# Autodesk Inventor assembly: Assembly
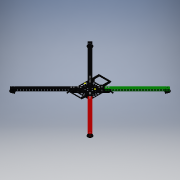
[picture p0: Inventor's stored thumbnail of the model, 180x180]
Saved by Autodesk Inventor 2016 (Build 200138000, 138)
## iProperties
Created: 2016-03-06
Part Number: Assembly
Document SubType Name: Assembly
Designer: dimas
Author: dimas
## Documents named in this file (10)
- C:\Users\dimas\Documents\lap_quad\Assembly.iam
- C:\Users\dimas\Documents\lap_quad\Arm_light.ipt
- C:\Users\dimas\Documents\lap_quad\frame_mount.ipt
- C:\Users\dimas\Documents\lap_quad\plate_mk2.ipt
- C:\Users\dimas\Documents\lap_quad\motor_mount.ipt
- C:\Users\dimas\Documents\lap_quad\battery_clip.ipt
- C:\Users\dimas\Documents\Inventor\Content Center Files\R2016\en-US\ANSI B18.3.1M(6)\ANSI B18.3.1M - M3x0.5 x 25(1).ipt
- C:\Users\dimas\Documents\Inventor\Content Center Files\R2016\en-US\AS 1971 (M - 6)\AS 1971 - 3.5(2).ipt
- C:\Users\dimas\Documents\Inventor\Content Center Files\R2016\en-US\AS 1112 (2)\AS 1112 - M3  Type 5.ipt
- C:\Users\dimas\Documents\Inventor\Content Center Files\R2016\en-US\AS 1112 (2)\AS 1112 - M3  Type 8.ipt
## Components (56 placed, 9 different names)
1. Arm_light:1 — Mate:1, Mate:2, Flush:1, Mate:25, Mate:26, Mate:27, Mate:40, Mate:41, Mate:66, Mate:67
2. frame_mount:1 — Mate:1, Mate:2, Flush:1, Mate:3, Mate:4, Flush:2, Mate:5, Mate:6, Flush:3, Mate:73, Mate:75
3. plate_mk2:1 — Mate:3, Mate:4, Flush:2, Mate:7, Mate:8, Mate:9, Mate:10, Mate:11, Mate:12, Mate:13, Mate:14, Mate:15, Flush:7, Flush:8, Flush:9, Mate:34, Mate:35, Mate:36, Mate:37, Mate:38, Mate:39, Mate:49, Mate:51, Mate:53, Mate:55, Mate:68, Mate:69, Mate:70, Mate:71
4. plate_mk2:2 — Mate:5, Mate:6, Flush:3, Mate:96
5. frame_mount:2 — Mate:7, Mate:8, Mate:9, Mate:16, Mate:17, Flush:4, Mate:77, Mate:79
6. frame_mount:3 — Mate:13, Mate:14, Mate:15, Mate:20, Mate:21, Flush:6, Mate:81, Mate:83
7. frame_mount:4 — Mate:10, Mate:11, Mate:12, Mate:18, Mate:19, Flush:5, Mate:85, Mate:87
8. Arm_light:2 — Mate:16, Mate:17, Flush:4, Mate:28, Mate:29, Mate:30, Mate:42, Mate:43, Mate:57, Mate:58
9. Arm_light:3 — Mate:18, Mate:19, Flush:5, Mate:31, Mate:32, Mate:33, Mate:46, Mate:47, Mate:63, Mate:64
10. Arm_light:4 — Mate:20, Mate:21, Flush:6, Mate:22, Mate:23, Mate:24, Mate:44, Mate:45, Mate:60, Mate:61
11. motor_mount:1 — Mate:22, Mate:23, Mate:24
12. motor_mount:2 — Mate:25, Mate:26, Mate:27
13. motor_mount:3 — Mate:28, Mate:29, Mate:30
14. motor_mount:4 — Mate:31, Mate:32, Mate:33
15. battery_clip:1 — Mate:34, Mate:35, Mate:36, Mate:48, Mate:54, Mate:59, Mate:62
16. battery_clip:2 — Mate:37, Mate:38, Mate:39, Mate:50, Mate:52, Mate:56, Mate:65
17. Forged Socket Head Cap Screw - Metric M3x0.5 x 25:1 — Mate:44, Mate:60, Mate:80, Mate:99
18. Forged Socket Head Cap Screw - Metric M3x0.5 x 25:2 — Mate:45, Mate:61, Mate:82, Mate:100
19. Forged Socket Head Cap Screw - Metric M3x0.5 x 25:3 — Mate:46, Mate:64, Mate:86, Mate:106
20. Forged Socket Head Cap Screw - Metric M3x0.5 x 25:4 — Mate:47, Mate:63, Mate:84, Mate:105
21. Forged Socket Head Cap Screw - Metric M3x0.5 x 25:5 — Mate:40, Mate:67, Mate:74, Mate:89
22. Forged Socket Head Cap Screw - Metric M3x0.5 x 25:6 — Mate:41, Mate:66, Mate:72, Mate:91
23. Forged Socket Head Cap Screw - Metric M3x0.5 x 25:7 — Mate:42, Mate:58, Mate:78, Mate:92
24. Forged Socket Head Cap Screw - Metric M3x0.5 x 25:8 — Mate:43, Mate:57, Mate:76, Mate:93
25. Forged Socket Head Cap Screw - Metric M3x0.5 x 25:9 — Mate:48, Mate:62, Mate:101
26. Forged Socket Head Cap Screw - Metric M3x0.5 x 25:10 — Mate:50, Mate:65, Mate:103
27. Forged Socket Head Cap Screw - Metric M3x0.5 x 25:11 — Mate:51, Mate:71, Mate:104
28. Forged Socket Head Cap Screw - Metric M3x0.5 x 25:12 — Mate:52, Mate:56, Mate:97
29. Forged Socket Head Cap Screw - Metric M3x0.5 x 25:13 — Mate:49, Mate:70, Mate:102
30. Forged Socket Head Cap Screw - Metric M3x0.5 x 25:14 — Mate:54, Mate:59, Mate:94
31. Forged Socket Head Cap Screw - Metric M3x0.5 x 25:15 — Mate:55, Mate:68, Mate:95
32. Forged Socket Head Cap Screw - Metric M3x0.5 x 25:16 — Mate:53, Mate:69, Mate:98
33. AS 1971 (M - 6) 3.5:1 — Mate:72, Mate:73
34. AS 1971 (M - 6) 3.5:2 — Mate:74, Mate:75, Mate:90
35. AS 1971 (M - 6) 3.5:3 — Mate:76, Mate:77
36. AS 1971 (M - 6) 3.5:4 — Mate:78, Mate:79
37. AS 1971 (M - 6) 3.5:5 — Mate:80, Mate:81
38. AS 1971 (M - 6) 3.5:6 — Mate:82, Mate:83
39. AS 1971 (M - 6) 3.5:7 — Mate:84, Mate:85
40. AS 1971 (M - 6) 3.5:8 — Mate:86, Mate:87
41. AS 1112 (2) - Metric M3  Type 5:1 — Mate:89, Mate:90, Flush:10, Flush:11, Flush:12, Flush:18
42. AS 1112 (2) - Metric M3  Type 8:1 — Mate:93, Flush:12
43. AS 1112 (2) - Metric M3  Type 8:2 — Mate:92, Flush:11
44. AS 1112 (2) - Metric M3  Type 8:3 — Mate:95, Flush:13, Flush:14, Flush:17
45. AS 1112 (2) - Metric M3  Type 8:4 — Mate:94, Mate:96, Flush:13, Flush:15, Flush:16
46. AS 1112 (2) - Metric M3  Type 8:5 — Mate:98, Flush:14
47. AS 1112 (2) - Metric M3  Type 8:6 — Mate:97, Flush:15
48. AS 1112 (2) - Metric M3  Type 8:7 — Mate:104, Flush:22, Flush:23
49. AS 1112 (2) - Metric M3  Type 8:8 — Mate:103, Flush:23
50. AS 1112 (2) - Metric M3  Type 8:9 — Mate:106, Flush:21
51. AS 1112 (2) - Metric M3  Type 8:10 — Mate:105, Flush:20, Flush:21
52. AS 1112 (2) - Metric M3  Type 8:11 — Mate:100, Flush:18, Flush:19, Flush:20
53. AS 1112 (2) - Metric M3  Type 8:12 — Mate:102, Flush:17, Flush:22
54. AS 1112 (2) - Metric M3  Type 8:13 — Mate:99, Flush:19
55. AS 1112 (2) - Metric M3  Type 8:14 — Mate:101, Flush:16
56. AS 1112 (2) - Metric M3  Type 8:15 — Mate:91, Flush:10
## Relationships (128: Mate 105, Flush 23)
- Mate:1: Arm_light:1 ↔ frame_mount:1
- Mate:2: Arm_light:1 ↔ frame_mount:1
- Flush:1: Arm_light:1 ↔ frame_mount:1
- Mate:3: frame_mount:1 ↔ plate_mk2:1
- Mate:4: frame_mount:1 ↔ plate_mk2:1
- Flush:2: frame_mount:1 ↔ plate_mk2:1
- Mate:5: frame_mount:1 ↔ plate_mk2:2
- Mate:6: frame_mount:1 ↔ plate_mk2:2
- Flush:3: frame_mount:1 ↔ plate_mk2:2
- Mate:7: plate_mk2:1 ↔ frame_mount:2
- Mate:8: plate_mk2:1 ↔ frame_mount:2
- Mate:9: plate_mk2:1 ↔ frame_mount:2
- Mate:10: plate_mk2:1 ↔ frame_mount:4
- Mate:11: plate_mk2:1 ↔ frame_mount:4
- Mate:12: plate_mk2:1 ↔ frame_mount:4
- Mate:13: plate_mk2:1 ↔ frame_mount:3
- Mate:14: plate_mk2:1 ↔ frame_mount:3
- Mate:15: plate_mk2:1 ↔ frame_mount:3
- Mate:16: frame_mount:2 ↔ Arm_light:2
- Mate:17: frame_mount:2 ↔ Arm_light:2
- Flush:4: frame_mount:2 ↔ Arm_light:2
- Mate:18: frame_mount:4 ↔ Arm_light:3
- Mate:19: frame_mount:4 ↔ Arm_light:3
- Flush:5: frame_mount:4 ↔ Arm_light:3
- Mate:20: frame_mount:3 ↔ Arm_light:4
- Mate:21: frame_mount:3 ↔ Arm_light:4
- Flush:6: frame_mount:3 ↔ Arm_light:4
- Flush:7: plate_mk2:1
- Flush:8: plate_mk2:1
- Flush:9: plate_mk2:1
- Mate:22: Arm_light:4 ↔ motor_mount:1
- Mate:23: Arm_light:4 ↔ motor_mount:1
- Mate:24: Arm_light:4 ↔ motor_mount:1
- Mate:25: Arm_light:1 ↔ motor_mount:2
- Mate:26: Arm_light:1 ↔ motor_mount:2
- Mate:27: Arm_light:1 ↔ motor_mount:2
- Mate:28: Arm_light:2 ↔ motor_mount:3
- Mate:29: Arm_light:2 ↔ motor_mount:3
- Mate:30: Arm_light:2 ↔ motor_mount:3
- Mate:31: Arm_light:3 ↔ motor_mount:4
- Mate:32: Arm_light:3 ↔ motor_mount:4
- Mate:33: Arm_light:3 ↔ motor_mount:4
- Mate:34: plate_mk2:1 ↔ battery_clip:1
- Mate:35: plate_mk2:1 ↔ battery_clip:1
- Mate:36: plate_mk2:1 ↔ battery_clip:1
- Mate:37: plate_mk2:1 ↔ battery_clip:2
- Mate:38: plate_mk2:1 ↔ battery_clip:2
- Mate:39: plate_mk2:1 ↔ battery_clip:2
- Mate:40: Arm_light:1 ↔ Forged Socket Head Cap Screw - Metric M3x0.5 x 25:5
- Mate:41: Arm_light:1 ↔ Forged Socket Head Cap Screw - Metric M3x0.5 x 25:6
- Mate:42: Arm_light:2 ↔ Forged Socket Head Cap Screw - Metric M3x0.5 x 25:7
- Mate:43: Arm_light:2 ↔ Forged Socket Head Cap Screw - Metric M3x0.5 x 25:8
- Mate:44: Arm_light:4 ↔ Forged Socket Head Cap Screw - Metric M3x0.5 x 25:1
- Mate:45: Arm_light:4 ↔ Forged Socket Head Cap Screw - Metric M3x0.5 x 25:2
- Mate:46: Arm_light:3 ↔ Forged Socket Head Cap Screw - Metric M3x0.5 x 25:3
- Mate:47: Arm_light:3 ↔ Forged Socket Head Cap Screw - Metric M3x0.5 x 25:4
- Mate:48: battery_clip:1 ↔ Forged Socket Head Cap Screw - Metric M3x0.5 x 25:9
- Mate:49: plate_mk2:1 ↔ Forged Socket Head Cap Screw - Metric M3x0.5 x 25:13
- Mate:50: battery_clip:2 ↔ Forged Socket Head Cap Screw - Metric M3x0.5 x 25:10
- Mate:51: plate_mk2:1 ↔ Forged Socket Head Cap Screw - Metric M3x0.5 x 25:11
- Mate:52: battery_clip:2 ↔ Forged Socket Head Cap Screw - Metric M3x0.5 x 25:12
- Mate:53: plate_mk2:1 ↔ Forged Socket Head Cap Screw - Metric M3x0.5 x 25:16
- Mate:54: battery_clip:1 ↔ Forged Socket Head Cap Screw - Metric M3x0.5 x 25:14
- Mate:55: plate_mk2:1 ↔ Forged Socket Head Cap Screw - Metric M3x0.5 x 25:15
- Mate:56: battery_clip:2 ↔ Forged Socket Head Cap Screw - Metric M3x0.5 x 25:12
- Mate:57: Arm_light:2 ↔ Forged Socket Head Cap Screw - Metric M3x0.5 x 25:8
- Mate:58: Arm_light:2 ↔ Forged Socket Head Cap Screw - Metric M3x0.5 x 25:7
- Mate:59: battery_clip:1 ↔ Forged Socket Head Cap Screw - Metric M3x0.5 x 25:14
- Mate:60: Arm_light:4 ↔ Forged Socket Head Cap Screw - Metric M3x0.5 x 25:1
- Mate:61: Arm_light:4 ↔ Forged Socket Head Cap Screw - Metric M3x0.5 x 25:2
- Mate:62: battery_clip:1 ↔ Forged Socket Head Cap Screw - Metric M3x0.5 x 25:9
- Mate:63: Arm_light:3 ↔ Forged Socket Head Cap Screw - Metric M3x0.5 x 25:4
- Mate:64: Arm_light:3 ↔ Forged Socket Head Cap Screw - Metric M3x0.5 x 25:3
- Mate:65: battery_clip:2 ↔ Forged Socket Head Cap Screw - Metric M3x0.5 x 25:10
- Mate:66: Arm_light:1 ↔ Forged Socket Head Cap Screw - Metric M3x0.5 x 25:6
- Mate:67: Arm_light:1 ↔ Forged Socket Head Cap Screw - Metric M3x0.5 x 25:5
- Mate:68: plate_mk2:1 ↔ Forged Socket Head Cap Screw - Metric M3x0.5 x 25:15
- Mate:69: plate_mk2:1 ↔ Forged Socket Head Cap Screw - Metric M3x0.5 x 25:16
- Mate:70: plate_mk2:1 ↔ Forged Socket Head Cap Screw - Metric M3x0.5 x 25:13
- Mate:71: plate_mk2:1 ↔ Forged Socket Head Cap Screw - Metric M3x0.5 x 25:11
- Mate:72: Forged Socket Head Cap Screw - Metric M3x0.5 x 25:6 ↔ AS 1971 (M - 6) 3.5:1
- Mate:73: frame_mount:1 ↔ AS 1971 (M - 6) 3.5:1
- Mate:74: Forged Socket Head Cap Screw - Metric M3x0.5 x 25:5 ↔ AS 1971 (M - 6) 3.5:2
- Mate:75: frame_mount:1 ↔ AS 1971 (M - 6) 3.5:2
- Mate:76: Forged Socket Head Cap Screw - Metric M3x0.5 x 25:8 ↔ AS 1971 (M - 6) 3.5:3
- Mate:77: frame_mount:2 ↔ AS 1971 (M - 6) 3.5:3
- Mate:78: Forged Socket Head Cap Screw - Metric M3x0.5 x 25:7 ↔ AS 1971 (M - 6) 3.5:4
- Mate:79: frame_mount:2 ↔ AS 1971 (M - 6) 3.5:4
- Mate:80: Forged Socket Head Cap Screw - Metric M3x0.5 x 25:1 ↔ AS 1971 (M - 6) 3.5:5
- Mate:81: frame_mount:3 ↔ AS 1971 (M - 6) 3.5:5
- Mate:82: Forged Socket Head Cap Screw - Metric M3x0.5 x 25:2 ↔ AS 1971 (M - 6) 3.5:6
- Mate:83: frame_mount:3 ↔ AS 1971 (M - 6) 3.5:6
- Mate:84: Forged Socket Head Cap Screw - Metric M3x0.5 x 25:4 ↔ AS 1971 (M - 6) 3.5:7
- Mate:85: frame_mount:4 ↔ AS 1971 (M - 6) 3.5:7
- Mate:86: Forged Socket Head Cap Screw - Metric M3x0.5 x 25:3 ↔ AS 1971 (M - 6) 3.5:8
- Mate:87: frame_mount:4 ↔ AS 1971 (M - 6) 3.5:8
- Mate:89: Forged Socket Head Cap Screw - Metric M3x0.5 x 25:5 ↔ AS 1112 (2) - Metric M3  Type 5:1
- Mate:90: AS 1971 (M - 6) 3.5:2 ↔ AS 1112 (2) - Metric M3  Type 5:1
- Mate:91: Forged Socket Head Cap Screw - Metric M3x0.5 x 25:6 ↔ AS 1112 (2) - Metric M3  Type 8:15
- Flush:10: AS 1112 (2) - Metric M3  Type 5:1 ↔ AS 1112 (2) - Metric M3  Type 8:15
- Mate:92: Forged Socket Head Cap Screw - Metric M3x0.5 x 25:7 ↔ AS 1112 (2) - Metric M3  Type 8:2
- Mate:93: Forged Socket Head Cap Screw - Metric M3x0.5 x 25:8 ↔ AS 1112 (2) - Metric M3  Type 8:1
- Flush:11: AS 1112 (2) - Metric M3  Type 5:1 ↔ AS 1112 (2) - Metric M3  Type 8:2
- Flush:12: AS 1112 (2) - Metric M3  Type 5:1 ↔ AS 1112 (2) - Metric M3  Type 8:1
- Mate:94: Forged Socket Head Cap Screw - Metric M3x0.5 x 25:14 ↔ AS 1112 (2) - Metric M3  Type 8:4
- Mate:95: Forged Socket Head Cap Screw - Metric M3x0.5 x 25:15 ↔ AS 1112 (2) - Metric M3  Type 8:3
- Mate:96: plate_mk2:2 ↔ AS 1112 (2) - Metric M3  Type 8:4
- Flush:13: AS 1112 (2) - Metric M3  Type 8:3 ↔ AS 1112 (2) - Metric M3  Type 8:4
- Mate:97: Forged Socket Head Cap Screw - Metric M3x0.5 x 25:12 ↔ AS 1112 (2) - Metric M3  Type 8:6
- Mate:98: Forged Socket Head Cap Screw - Metric M3x0.5 x 25:16 ↔ AS 1112 (2) - Metric M3  Type 8:5
- Flush:14: AS 1112 (2) - Metric M3  Type 8:3 ↔ AS 1112 (2) - Metric M3  Type 8:5
- Flush:15: AS 1112 (2) - Metric M3  Type 8:4 ↔ AS 1112 (2) - Metric M3  Type 8:6
- Mate:99: Forged Socket Head Cap Screw - Metric M3x0.5 x 25:1 ↔ AS 1112 (2) - Metric M3  Type 8:13
- Mate:100: Forged Socket Head Cap Screw - Metric M3x0.5 x 25:2 ↔ AS 1112 (2) - Metric M3  Type 8:11
- Mate:101: Forged Socket Head Cap Screw - Metric M3x0.5 x 25:9 ↔ AS 1112 (2) - Metric M3  Type 8:14
- Mate:102: Forged Socket Head Cap Screw - Metric M3x0.5 x 25:13 ↔ AS 1112 (2) - Metric M3  Type 8:12
- Flush:16: AS 1112 (2) - Metric M3  Type 8:4 ↔ AS 1112 (2) - Metric M3  Type 8:14
- Flush:17: AS 1112 (2) - Metric M3  Type 8:3 ↔ AS 1112 (2) - Metric M3  Type 8:12
- Flush:18: AS 1112 (2) - Metric M3  Type 5:1 ↔ AS 1112 (2) - Metric M3  Type 8:11
- Flush:19: AS 1112 (2) - Metric M3  Type 8:11 ↔ AS 1112 (2) - Metric M3  Type 8:13
- Mate:103: Forged Socket Head Cap Screw - Metric M3x0.5 x 25:10 ↔ AS 1112 (2) - Metric M3  Type 8:8
- Mate:104: Forged Socket Head Cap Screw - Metric M3x0.5 x 25:11 ↔ AS 1112 (2) - Metric M3  Type 8:7
- Mate:105: Forged Socket Head Cap Screw - Metric M3x0.5 x 25:4 ↔ AS 1112 (2) - Metric M3  Type 8:10
- Mate:106: Forged Socket Head Cap Screw - Metric M3x0.5 x 25:3 ↔ AS 1112 (2) - Metric M3  Type 8:9
- Flush:20: AS 1112 (2) - Metric M3  Type 8:10 ↔ AS 1112 (2) - Metric M3  Type 8:11
- Flush:21: AS 1112 (2) - Metric M3  Type 8:9 ↔ AS 1112 (2) - Metric M3  Type 8:10
- Flush:22: AS 1112 (2) - Metric M3  Type 8:7 ↔ AS 1112 (2) - Metric M3  Type 8:12
- Flush:23: AS 1112 (2) - Metric M3  Type 8:7 ↔ AS 1112 (2) - Metric M3  Type 8:8
